# Autodesk Inventor assembly: victor
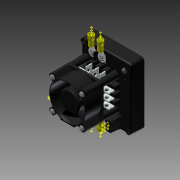
[picture p0: Inventor's stored thumbnail of the model, 180x180]
Saved by Autodesk Inventor 2011 (Build 150239000, 239)
## iProperties
Created: 2010-02-13
Part Number: victor
Document SubType Name: Assembly
Designer: a
Author: a
## Documents named in this file (3)
- R:\2012\Inventor\vkop\All-Control-System\victor.iam
- R:\2012\Inventor\vkop\All-Control-System\Control System_Innovation First_FR-VIC884.ipt
- R:\2012\Inventor\vkop\All-Electrical\RingTerminal_Tyco_320619_yellow.ipt
## Components (5 placed, 2 different names)
1. Control System_Innovation First_FR-VIC884:1 — Mate:1, Mate:2, Mate:3, Mate:4, Mate:5, Mate:6, Mate:7, Mate:8, Angle:1, Angle:2, Angle:3, Angle:4
2. RingTerminal_Tyco_320619_yellow:1 — Mate:5, Mate:6, Angle:1
3. RingTerminal_Tyco_320619_yellow:2 — Mate:7, Mate:8, Angle:2
4. RingTerminal_Tyco_320619_yellow:3 — Mate:1, Mate:3, Angle:3
5. RingTerminal_Tyco_320619_yellow:4 — Mate:2, Mate:4, Angle:4
## Relationships (12: Mate 8, Angle 4)
- Mate:1: Control System_Innovation First_FR-VIC884:1 ↔ RingTerminal_Tyco_320619_yellow:3
- Mate:2: Control System_Innovation First_FR-VIC884:1 ↔ RingTerminal_Tyco_320619_yellow:4
- Mate:3: Control System_Innovation First_FR-VIC884:1 ↔ RingTerminal_Tyco_320619_yellow:3
- Mate:4: Control System_Innovation First_FR-VIC884:1 ↔ RingTerminal_Tyco_320619_yellow:4
- Mate:5: Control System_Innovation First_FR-VIC884:1 ↔ RingTerminal_Tyco_320619_yellow:1
- Mate:6: Control System_Innovation First_FR-VIC884:1 ↔ RingTerminal_Tyco_320619_yellow:1
- Mate:7: Control System_Innovation First_FR-VIC884:1 ↔ RingTerminal_Tyco_320619_yellow:2
- Mate:8: Control System_Innovation First_FR-VIC884:1 ↔ RingTerminal_Tyco_320619_yellow:2
- Angle:1 (0 deg): Control System_Innovation First_FR-VIC884:1 ↔ RingTerminal_Tyco_320619_yellow:1
- Angle:2 (0 deg): Control System_Innovation First_FR-VIC884:1 ↔ RingTerminal_Tyco_320619_yellow:2
- Angle:3 (0 deg): Control System_Innovation First_FR-VIC884:1 ↔ RingTerminal_Tyco_320619_yellow:3
- Angle:4 (0 deg): Control System_Innovation First_FR-VIC884:1 ↔ RingTerminal_Tyco_320619_yellow:4
